# Autodesk Inventor assembly: zloz_2
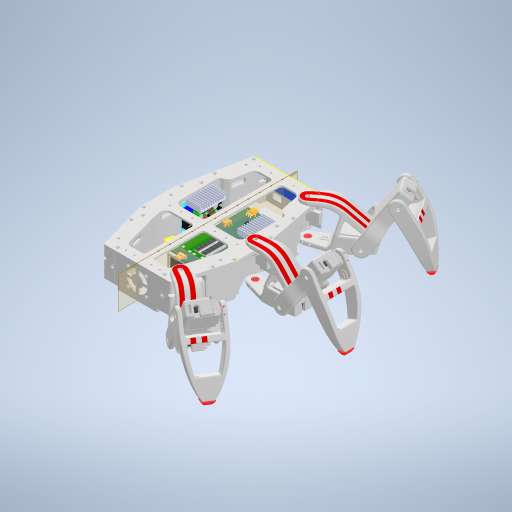
[picture p0: Inventor's stored thumbnail of the model, 512x512]
Saved by Autodesk Inventor 2023.4 (Build 274418000, 418)
## iProperties
Created: 2024-07-26
Part Number: zloz_2
Document SubType Name: Assembly
Designer: kamil
Author: kamil
## Documents named in this file (15)
- E:\PROJECTS_REPOS\Robal-2.0\mechanics\zloz_2.iam
- E:\PROJECTS_REPOS\Robal-2.0\mechanics\Sub-Assy Buck Converter.ipt
- E:\PROJECTS_REPOS\Robal-2.0\mechanics\li_pol_3S_5000mAh.ipt
- E:\PROJECTS_REPOS\Robal-2.0\mechanics\uchwyt_serwa_podwojny.ipt
- E:\PROJECTS_REPOS\Robal-2.0\mechanics\uchwyt_serwa_podwojny_MIR.ipt
- E:\PROJECTS_REPOS\Robal-2.0\mechanics\dol.ipt
- E:\PROJECTS_REPOS\Robal-2.0\mechanics\gora.ipt
- E:\PROJECTS_REPOS\Robal-2.0\mechanics\Lithium Battery Capacity Indicator Module.ipt
- E:\PROJECTS_REPOS\Robal-2.0\mechanics\pokrywa_tyl.ipt
- E:\PROJECTS_REPOS\Robal-2.0\mechanics\pokrywa_przod.ipt
- E:\PROJECTS_REPOS\Robal-2.0\mechanics\noga_pre.iam
- E:\PROJECTS_REPOS\Robal-2.0\mechanics\Standard-Servo.ipt
- E:\PROJECTS_REPOS\Robal-2.0\mechanics\uchwyt_li_pol.ipt
- E:\PROJECTS_REPOS\Robal-2.0\mechanics\robal_power_board_6.ipt
- E:\PROJECTS_REPOS\Robal-2.0\mechanics\pokrywa_gora.ipt
## Components (17 placed, 14 different names)
1. Sub-Assy Buck Converter:1 — Mate:20, Mate:24, Mate:25
2. li_pol_3S_5000mAh:1 — Zestawiające:48, Zestawiające:49
3. uchwyt_serwa_podwojny:1 — Mate:14, Mate:15, Mate:16, Mate:20, Mate:21, Mate:24, Mate:25, Mate:32, Flush:13, Mate:33, Równoległe:14, Symetria:1
4. uchwyt_serwa_podwojny_MIR:1 — Mate:17, Mate:22, Mate:23, Mate:26, Mate:27, Mate:28, Mate:30, Mate:31, Mate:34, Mate:38, Angle:1, Mate:44, Mate:45, Symetria:1
5. dol:1 — Mate:11, Mate:12, Mate:13, Mate:14, Mate:15, Mate:16, Mate:17, Zestawiające:48
6. gora:1 — Mate:21, Mate:22, Mate:23, Mate:39, Mate:40, Mate:41, Mate:42, Mate:43, Równoległe:14, Zestawiające:53, Zestawiające:54
7. Lithium Battery Capacity Indicator Module:1 — Mate:35, Mate:36, Mate:37
8. Sub-Assy Buck Converter:2 — Mate:26, Mate:27, Mate:28
9. pokrywa_tyl:1 — Mate:30, Mate:31, Mate:32, Mate:35, Mate:36, Mate:37, Równoległe:15
10. pokrywa_przod:1 — Flush:13, Mate:33, Mate:34
11. noga_pre:1 [sub-assembly] — Mate:38, Mate:39, Mate:46
12. noga_pre:2 [sub-assembly] — Mate:40, Mate:41
13. noga_pre:3 [sub-assembly] — Mate:42, Mate:43
14. Standard-Servo:1 — Angle:1, Mate:44, Mate:45, Mate:46
15. uchwyt_li_pol:1 — Zestawiające:49, Zestawiające:50, Zestawiające:51, Zestawiające:52
16. robal_power_board_6:1 — Zestawiające:50, Zestawiające:51, Zestawiające:52
17. pokrywa_gora:1 — Równoległe:15, Zestawiające:53, Zestawiające:54
## Relationships (45: Mate 40, Flush 3, Angle 1, Symmetry 1)
- Mate:11 (-31.7995 mm): dol:1
- Mate:12: dol:1
- Mate:13: dol:1
- Mate:14: uchwyt_serwa_podwojny:1 ↔ dol:1
- Mate:15: uchwyt_serwa_podwojny:1 ↔ dol:1
- Mate:16: uchwyt_serwa_podwojny:1 ↔ dol:1
- Mate:17: uchwyt_serwa_podwojny_MIR:1 ↔ dol:1
- Mate:20: Sub-Assy Buck Converter:1 ↔ uchwyt_serwa_podwojny:1
- Mate:21: uchwyt_serwa_podwojny:1 ↔ gora:1
- Mate:22: uchwyt_serwa_podwojny_MIR:1 ↔ gora:1
- Mate:23: uchwyt_serwa_podwojny_MIR:1 ↔ gora:1
- Mate:24: Sub-Assy Buck Converter:1 ↔ uchwyt_serwa_podwojny:1
- Mate:25: Sub-Assy Buck Converter:1 ↔ uchwyt_serwa_podwojny:1
- Mate:26: uchwyt_serwa_podwojny_MIR:1 ↔ Sub-Assy Buck Converter:2
- Mate:27: uchwyt_serwa_podwojny_MIR:1 ↔ Sub-Assy Buck Converter:2
- Mate:28: uchwyt_serwa_podwojny_MIR:1 ↔ Sub-Assy Buck Converter:2
- Mate:30 (0.1 mm): uchwyt_serwa_podwojny_MIR:1 ↔ pokrywa_tyl:1
- Mate:31: uchwyt_serwa_podwojny_MIR:1 ↔ pokrywa_tyl:1
- Mate:32: uchwyt_serwa_podwojny:1 ↔ pokrywa_tyl:1
- Flush:13: uchwyt_serwa_podwojny:1 ↔ pokrywa_przod:1
- Mate:33: uchwyt_serwa_podwojny:1 ↔ pokrywa_przod:1
- Mate:34: uchwyt_serwa_podwojny_MIR:1 ↔ pokrywa_przod:1
- Mate:35: Lithium Battery Capacity Indicator Module:1 ↔ pokrywa_tyl:1
- Mate:36: Lithium Battery Capacity Indicator Module:1 ↔ pokrywa_tyl:1
- Mate:37: Lithium Battery Capacity Indicator Module:1 ↔ pokrywa_tyl:1
- Mate:38: uchwyt_serwa_podwojny_MIR:1 ↔ noga_pre:1
- Mate:39: gora:1 ↔ noga_pre:1
- Mate:40: gora:1 ↔ noga_pre:2
- Mate:41: gora:1 ↔ noga_pre:2
- Mate:42: gora:1 ↔ noga_pre:3
- Mate:43: gora:1 ↔ noga_pre:3
- Angle:1 (180 deg): uchwyt_serwa_podwojny_MIR:1 ↔ Standard-Servo:1
- Mate:44: uchwyt_serwa_podwojny_MIR:1 ↔ Standard-Servo:1
- Mate:45: uchwyt_serwa_podwojny_MIR:1 ↔ Standard-Servo:1
- Mate:46: noga_pre:1 ↔ Standard-Servo:1
- Równoległe:14 [Flush]: uchwyt_serwa_podwojny:1 ↔ gora:1
- Symetria:1 [Symmetry]: uchwyt_serwa_podwojny:1 ↔ uchwyt_serwa_podwojny_MIR:1
- Zestawiające:48 [Mate]: li_pol_3S_5000mAh:1 ↔ dol:1
- Zestawiające:49 [Mate]: li_pol_3S_5000mAh:1 ↔ uchwyt_li_pol:1
- Zestawiające:50 [Mate]: uchwyt_li_pol:1 ↔ robal_power_board_6:1
- Zestawiające:51 [Mate]: uchwyt_li_pol:1 ↔ robal_power_board_6:1
- Zestawiające:52 [Mate]: uchwyt_li_pol:1 ↔ robal_power_board_6:1
- Równoległe:15 [Flush]: pokrywa_tyl:1 ↔ pokrywa_gora:1
- Zestawiające:53 [Mate]: gora:1 ↔ pokrywa_gora:1
- Zestawiające:54 [Mate]: gora:1 ↔ pokrywa_gora:1
